# Autodesk Inventor assembly: Arm
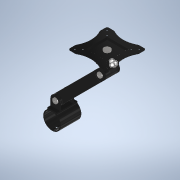
[picture p0: Inventor's stored thumbnail of the model, 180x180]
Saved by Autodesk Inventor 2020 (Build 240168000, 168)
## iProperties
Created: 2021-07-08
Part Number: Arm
Document SubType Name: Assembly
Designer: Simon.Alvarez
Author: Simon.Alvarez
## Documents named in this file (8)
- C:\Users\Simon.Alvarez\Desktop\Simon off laptop\Desk\Monitor Stand\Arm.iam
- C:\Users\Simon.Alvarez\Desktop\Simon off laptop\Desk\Monitor Stand\Hanger_Clamp.ipt
- C:\Users\Simon.Alvarez\Desktop\Simon off laptop\Desk\Monitor Stand\Bearing.ipt
- C:\Users\Simon.Alvarez\Documents\Inventor\Content Center Files\R2020\en-US\BS EN ISO 7045 Z\EN ISO 7045 - M8 x 12 - 4.8 - Z(1).ipt
- C:\Users\Simon.Alvarez\Desktop\Simon off laptop\Desk\Monitor Stand\Hinge.ipt
- C:\Users\Simon.Alvarez\Desktop\Simon off laptop\Desk\Monitor Stand\Swivel.ipt
- C:\Users\Simon.Alvarez\Desktop\Simon off laptop\Desk\Monitor Stand\Plate.ipt
- C:\Users\Simon.Alvarez\Documents\Inventor\Content Center Files\R2020\en-US\GB 833-88\Screw GB 833 M6 x 10.ipt
## Components (13 placed, 7 different names)
1. Hanger_Clamp:1 — Flush:1, Flush:2, Flush:3, Mate:1, Mate:2, Mate:3, Mate:4, Mate:5, Mate:6, Angle:1
2. Bearing:1 — Mate:1, Mate:2, Mate:7, Mate:8, Flush:4, Angle:1, Angle:2
3. BS EN ISO 7045 Z - Metric M8 x 12 - 4.8 - Z:1 — Mate:3, Mate:4
4. BS EN ISO 7045 Z - Metric M8 x 12 - 4.8 - Z:2 — Mate:5, Mate:6
5. Hinge:1 — Mate:7, Mate:8, Flush:4, Mate:9, Mate:10, Mate:13, Mate:14, Mate:15, Mate:16
6. Swivel:1 — Mate:9, Mate:10, Mate:11, Mate:12, Angle:2
7. Hinge:2 — Mate:11, Mate:12, Mate:17, Mate:18, Mate:19, Mate:20, Mate:21, Mate:22, Angle:3, Angle:4
8. BS EN ISO 7045 Z - Metric M8 x 12 - 4.8 - Z:3 — Mate:13, Mate:14
9. BS EN ISO 7045 Z - Metric M8 x 12 - 4.8 - Z:4 — Mate:15, Mate:16
10. BS EN ISO 7045 Z - Metric M8 x 12 - 4.8 - Z:5 — Mate:17, Mate:18
11. BS EN ISO 7045 Z - Metric M8 x 12 - 4.8 - Z:6 — Mate:19, Mate:20
12. Plate:1 — Mate:21, Mate:22, Angle:4, Mate:23, Mate:24
13. Screw GB/T 833-1988 M6 x 10:1 — Mate:23, Mate:24
## Relationships (32: Mate 24, Flush 4, Angle 4)
- Flush:1: Hanger_Clamp:1
- Flush:2: Hanger_Clamp:1
- Flush:3: Hanger_Clamp:1
- Mate:1: Hanger_Clamp:1 ↔ Bearing:1
- Mate:2: Hanger_Clamp:1 ↔ Bearing:1
- Mate:3: Hanger_Clamp:1 ↔ BS EN ISO 7045 Z - Metric M8 x 12 - 4.8 - Z:1
- Mate:4: Hanger_Clamp:1 ↔ BS EN ISO 7045 Z - Metric M8 x 12 - 4.8 - Z:1
- Mate:5: Hanger_Clamp:1 ↔ BS EN ISO 7045 Z - Metric M8 x 12 - 4.8 - Z:2
- Mate:6: Hanger_Clamp:1 ↔ BS EN ISO 7045 Z - Metric M8 x 12 - 4.8 - Z:2
- Mate:7: Bearing:1 ↔ Hinge:1
- Mate:8: Bearing:1 ↔ Hinge:1
- Flush:4 (-6.5 mm): Bearing:1 ↔ Hinge:1
- Mate:9: Hinge:1 ↔ Swivel:1
- Mate:10: Hinge:1 ↔ Swivel:1
- Mate:11: Swivel:1 ↔ Hinge:2
- Mate:12: Swivel:1 ↔ Hinge:2
- Mate:13: Hinge:1 ↔ BS EN ISO 7045 Z - Metric M8 x 12 - 4.8 - Z:3
- Mate:14: Hinge:1 ↔ BS EN ISO 7045 Z - Metric M8 x 12 - 4.8 - Z:3
- Mate:15: Hinge:1 ↔ BS EN ISO 7045 Z - Metric M8 x 12 - 4.8 - Z:4
- Mate:16: Hinge:1 ↔ BS EN ISO 7045 Z - Metric M8 x 12 - 4.8 - Z:4
- Mate:17: Hinge:2 ↔ BS EN ISO 7045 Z - Metric M8 x 12 - 4.8 - Z:5
- Mate:18: Hinge:2 ↔ BS EN ISO 7045 Z - Metric M8 x 12 - 4.8 - Z:5
- Mate:19: Hinge:2 ↔ BS EN ISO 7045 Z - Metric M8 x 12 - 4.8 - Z:6
- Mate:20: Hinge:2 ↔ BS EN ISO 7045 Z - Metric M8 x 12 - 4.8 - Z:6
- Mate:21: Hinge:2 ↔ Plate:1
- Mate:22: Hinge:2 ↔ Plate:1
- Angle:1 (-45 deg): Hanger_Clamp:1 ↔ Bearing:1
- Angle:2 (-135 deg): Bearing:1 ↔ Swivel:1
- Angle:3 (0 deg): Hinge:2
- Angle:4 (0 deg): Hinge:2 ↔ Plate:1
- Mate:23: Plate:1 ↔ Screw GB/T 833-1988 M6 x 10:1
- Mate:24: Plate:1 ↔ Screw GB/T 833-1988 M6 x 10:1
